# Autodesk Inventor assembly: A2017_T2_01
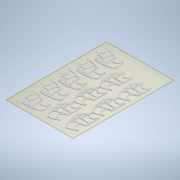
[picture p0: Inventor's stored thumbnail of the model, 180x180]
Saved by Autodesk Inventor 2022 (Build 260153000, 153)
## iProperties
Created: 2022-09-28
Part Number: A2017_T2_01
Document SubType Name: Assembly
Designer: Masato
Author: Masato
## Documents named in this file (3)
- C:\Users\6343y\ドキュメント\Inventor\SUSTAINA-OP\Cam\A2017_T2\A2017_T2_01.iam
- C:\Users\6343y\ドキュメント\Inventor\SUSTAINA-OP\Cam\DisposableBoard.ipt
- C:\Users\6343y\ドキュメント\Inventor\SUSTAINA-OP\LowerBody\Knee\Knee_side_frame.ipt
## Components (12 placed, 2 different names)
1. DisposableBoard:1 — フラッシュ:1, フラッシュ:2, フラッシュ:3, フラッシュ:4, フラッシュ:5, 正接:1, フラッシュ:6, 正接:2
2. Knee_side_frame:1 — メイト:1, フラッシュ:5, 正接:1
3. Knee_side_frame:2
4. Knee_side_frame:3
5. Knee_side_frame:4
6. Knee_side_frame:5
7. Knee_side_frame:6 — メイト:2, フラッシュ:6, 正接:2
8. Knee_side_frame:7
9. Knee_side_frame:8
10. Knee_side_frame:9
11. Knee_side_frame:10
12. Knee_side_frame:11
## Component patterns: (5 elements, first: Knee_side_frame:1), (6 elements, first: Knee_side_frame:6)
## Relationships (10: Flush 6, Mate 2, Tangent 2)
- フラッシュ:1 [Flush]: DisposableBoard:1
- フラッシュ:2 [Flush]: DisposableBoard:1
- フラッシュ:3 [Flush]: DisposableBoard:1
- フラッシュ:4 [Flush]: DisposableBoard:1
- メイト:1 [Mate]: Knee_side_frame:1
- フラッシュ:5 [Flush] (2.1 mm): DisposableBoard:1 ↔ Knee_side_frame:1
- 正接:1 [Tangent] (2.1 mm): DisposableBoard:1 ↔ Knee_side_frame:1
- メイト:2 [Mate]: Knee_side_frame:6
- フラッシュ:6 [Flush] (-2.1 mm): DisposableBoard:1 ↔ Knee_side_frame:6
- 正接:2 [Tangent] (2.1 mm): DisposableBoard:1 ↔ Knee_side_frame:6
